# Autodesk Inventor assembly: Maszyna1
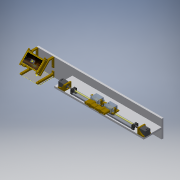
[picture p0: Inventor's stored thumbnail of the model, 180x180]
Saved by Autodesk Inventor 2019 (Build 230136000, 136)
## iProperties
Created: 2021-10-06
Part Number: Maszyna1
Document SubType Name: Assembly
Designer: Pokick
Author: Pokick
## Documents named in this file (23)
- C:\Users\Pokick\Desktop\PWR\SEM7\INZYNIER\maszyna\Maszyna1.iam
- C:\Users\Pokick\Desktop\PWR\SEM7\INZYNIER\maszyna\nema11_SY28STH32-0674A.ipt
- C:\Users\Pokick\Desktop\PWR\SEM7\INZYNIER\maszyna\LF20MG.ipt
- C:\Users\Pokick\Desktop\PWR\SEM7\INZYNIER\maszyna\Nema11_holder.ipt
- C:\Users\Pokick\Desktop\PWR\SEM7\INZYNIER\maszyna\LF20MG_MIR.ipt
- C:\Users\Pokick\Desktop\PWR\SEM7\INZYNIER\maszyna\back_plate.ipt
- C:\Users\Pokick\Desktop\PWR\SEM7\INZYNIER\maszyna\basePlate.ipt
- C:\Users\Pokick\Desktop\PWR\SEM7\INZYNIER\maszyna\raspberry_test.iam
- C:\Users\Pokick\Desktop\PWR\SEM7\INZYNIER\maszyna\orczyk_powerHD.ipt
- C:\Users\Pokick\Desktop\PWR\SEM7\INZYNIER\maszyna\orczyk_powerHD_MIR.ipt
- C:\Users\Pokick\Desktop\PWR\SEM7\INZYNIER\maszyna\PCB.ipt
- C:\Users\Pokick\Desktop\PWR\SEM7\INZYNIER\maszyna\PCB_STAND.ipt
- C:\Users\Pokick\Desktop\PWR\SEM7\INZYNIER\maszyna\sample_holder_v1.1.ipt
- C:\Users\Pokick\Desktop\PWR\SEM7\INZYNIER\maszyna\sample_holder_v1.1_MIR.ipt
- C:\Users\Pokick\Desktop\PWR\SEM7\INZYNIER\maszyna\big_servo_hold.ipt
- C:\Users\Pokick\Desktop\PWR\SEM7\INZYNIER\maszyna\SLNV_27_100_2.ipt
- C:\Users\Pokick\Desktop\PWR\SEM7\INZYNIER\maszyna\sample_hold_v2.ipt
- C:\Users\Pokick\Desktop\PWR\SEM7\INZYNIER\maszyna\nema11.ipt
- C:\Users\Pokick\Desktop\PWR\SEM7\INZYNIER\maszyna\Nema11_holder_MIR.ipt
- C:\Users\Pokick\Desktop\PWR\SEM7\INZYNIER\maszyna\big_servo_hold_MIR.ipt
- C:\Users\Pokick\Desktop\PWR\SEM7\INZYNIER\maszyna\SLNV_27_100_2_MIR.ipt
- C:\Users\Pokick\Desktop\PWR\SEM7\INZYNIER\maszyna\sample_hold_v2_MIR.ipt
- C:\Users\Pokick\Desktop\PWR\SEM7\INZYNIER\maszyna\nema11_MIR.ipt
## Components (28 placed, 22 different names)
1. LF20MG_MIR:1
2. back_plate:1 — Flush:8, Flush:12, Mate:4, Mate:5
3. basePlate:1 — Flush:8, Flush:9, Flush:10, Mate:1, Mate:2, Mate:3, Flush:12
4. raspberry_test:1 [sub-assembly] — Flush:9, Flush:10
5. LF20MG:1 — Rigid:8
6. orczyk_powerHD:1 — Rigid:8
7. orczyk_powerHD_MIR:1 — Rigid:11, Flush:11
8. LF20MG:2 — Rigid:11
9. PCB:1 — Rigid:9, Rigid:10
10. PCB_STAND:1 — Rigid:10
11. PCB_STAND:2 — Rigid:9, Mate:1, Mate:2, Mate:3
12. sample_holder_v1.1:1 — Flush:11
13. sample_holder_v1.1_MIR:1
14. Nema11_holder:1 — Mate:4, Mate:5, Rotational:1
15. nema11_SY28STH32-0674A:1 — Rotational:1, Rigid:12
16. big_servo_hold:1 — Rigid:13, Rotational:2
17. SLNV_27_100_2:1 — Rigid:12, Rigid:13, Rigid:15
18. LF20MG:3 — Rotational:2, Rigid:14
19. orczyk_powerHD:2 — Rigid:14, Flush:13
20. sample_hold_v2:1 — Flush:13
21. nema11:1 — Rigid:15
22. Nema11_holder_MIR:1
23. big_servo_hold_MIR:1 — Rigid:16
24. SLNV_27_100_2_MIR:1
25. LF20MG_MIR:2
26. sample_hold_v2_MIR:1
27. nema11_MIR:1
28. LF20MG:4 — Rigid:16
## Relationships (22: WeldJoint 9, Flush 6, Mate 5, RevoluteJoint 2)
- Flush:8: back_plate:1 ↔ basePlate:1
- Flush:9: basePlate:1 ↔ raspberry_test:1
- Flush:10: basePlate:1 ↔ raspberry_test:1
- Rigid:8 [WeldJoint]: LF20MG:1 ↔ orczyk_powerHD:1
- Rigid:9 [WeldJoint]: PCB:1 ↔ PCB_STAND:2
- Rigid:10 [WeldJoint]: PCB:1 ↔ PCB_STAND:1
- Mate:1: basePlate:1 ↔ PCB_STAND:2
- Mate:2: basePlate:1 ↔ PCB_STAND:2
- Mate:3: basePlate:1 ↔ PCB_STAND:2
- Rigid:11 [WeldJoint]: orczyk_powerHD_MIR:1 ↔ LF20MG:2
- Flush:11: orczyk_powerHD_MIR:1 ↔ sample_holder_v1.1:1
- Flush:12: back_plate:1 ↔ basePlate:1
- Mate:4: back_plate:1 ↔ Nema11_holder:1
- Mate:5: back_plate:1 ↔ Nema11_holder:1
- Rotational:1 [RevoluteJoint]: Nema11_holder:1 ↔ nema11_SY28STH32-0674A:1
- Rigid:12 [WeldJoint]: nema11_SY28STH32-0674A:1 ↔ SLNV_27_100_2:1
- Rigid:13 [WeldJoint]: big_servo_hold:1 ↔ SLNV_27_100_2:1
- Rotational:2 [RevoluteJoint]: big_servo_hold:1 ↔ LF20MG:3
- Rigid:14 [WeldJoint]: LF20MG:3 ↔ orczyk_powerHD:2
- Flush:13: orczyk_powerHD:2 ↔ sample_hold_v2:1
- Rigid:15 [WeldJoint]: SLNV_27_100_2:1 ↔ nema11:1
- Rigid:16 [WeldJoint]: big_servo_hold_MIR:1 ↔ LF20MG:4
